# Autodesk Inventor assembly: ElevatorClaw
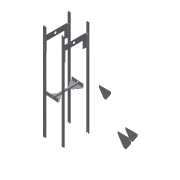
[picture p0: Inventor's stored thumbnail of the model, 180x180]
Saved by Autodesk Inventor 2015 (Build 190159000, 159)
## iProperties
Created: 2015-01-10
Part Number: ElevatorClaw
Document SubType Name: Assembly
Designer: Tanner
Author: Tanner
## Documents named in this file (8)
- C:\Users\Tanner\Documents\GitHub\FIRST-Team-1719-CAD-Team\2015 Robot CAD\Devices\Elevator and Claw\ElevatorClaw.iam
- C:\Users\Tanner\Documents\Inventor\ElevatorCAD\Kevin'sCustomUnistrut.ipt
- C:\Users\Tanner\Documents\Inventor\ElevatorCAD\Elevatorcarv2.iam
- C:\Users\Tanner\Documents\Inventor\ElevatorCAD\CarLbraket.ipt
- C:\Users\Tanner\Documents\Inventor\ElevatorCAD\elevbackplt.ipt
- C:\Users\Tanner\Documents\Inventor\ElevatorCAD\1 by 1 for the middle part of the elevator i dont even care anymore about names.ipt
- C:\Users\Tanner\Documents\Inventor\ElevatorCAD\super2.ipt
- C:\Users\Tanner\Documents\Inventor\ElevatorCAD\super4.ipt
## Components (21 placed, 7 different names)
1. Kevin'sCustomUnistrut:2 — Flush:17, Flush:27, Flush:28, Tangent:1, Mate:10
2. Kevin'sCustomUnistrut:3 — Flush:17, Flush:27, Flush:28, Tangent:2, Mate:11, Flush:48, Flush:51
3. Elevatorcarv2:1 [sub-assembly] — Flush:32, Mate:7, Flush:33, Tangent:2, Mate:11
4. Elevatorcarv2:3 [sub-assembly] — Mate:2, Flush:25, Flush:34, Tangent:1, Mate:10
5. CarLbraket:1 — Mate:2, Flush:25, Mate:4, Flush:34, Mate:9, Flush:37
6. CarLbraket:2 — Mate:4, Flush:32, Mate:7, Flush:33, Mate:8, Flush:35, Flush:36
7. elevbackplt:1 — Mate:8, Mate:9, Flush:35, Flush:36, Flush:37
8. Kevin'sCustomUnistrut:4
9. Kevin'sCustomUnistrut:5
10. Elevatorcarv2:4 [sub-assembly]
11. Elevatorcarv2:5 [sub-assembly]
12. CarLbraket:3
13. CarLbraket:4
14. elevbackplt:2
15. 1 by 1 for the middle part of the elevator i dont even care anymore about names:1 — Flush:48, Flush:49, Mate:19, Mate:20, Flush:50, Mate:21, Mate:22
16. super2:1 — Flush:50, Mate:21, Flush:51, Mate:22
17. super2:2 — Flush:49, Mate:19, Mate:20
18. super4:2
19. super4:4
20. super4:6
21. super4:9
## Relationships (46: Flush 24, Mate 18, Tangent 4)
- Flush:17: Kevin'sCustomUnistrut:2 ↔ Kevin'sCustomUnistrut:3
- Mate:2: Elevatorcarv2:3 ↔ CarLbraket:1
- Flush:25: Elevatorcarv2:3 ↔ CarLbraket:1
- Flush:27: Kevin'sCustomUnistrut:2 ↔ Kevin'sCustomUnistrut:3
- Flush:28: Kevin'sCustomUnistrut:2 ↔ Kevin'sCustomUnistrut:3
- Mate:4 (432.7144 mm): CarLbraket:1 ↔ CarLbraket:2
- Flush:32: Elevatorcarv2:1 ↔ CarLbraket:2
- Mate:7: Elevatorcarv2:1 ↔ CarLbraket:2
- Flush:33: Elevatorcarv2:1 ↔ CarLbraket:2
- Flush:34: Elevatorcarv2:3 ↔ CarLbraket:1
- Mate:8: CarLbraket:2 ↔ elevbackplt:1
- Mate:9: CarLbraket:1 ↔ elevbackplt:1
- Flush:35: CarLbraket:2 ↔ elevbackplt:1
- Flush:36 (-1.3462 mm): CarLbraket:2 ↔ elevbackplt:1
- Flush:37: CarLbraket:1 ↔ elevbackplt:1
- Tangent:1: Kevin'sCustomUnistrut:2 ↔ Elevatorcarv2:3
- Mate:10 (0.3683 mm): Kevin'sCustomUnistrut:2 ↔ Elevatorcarv2:3
- Tangent:2: Kevin'sCustomUnistrut:3 ↔ Elevatorcarv2:1
- Mate:11 (0.3683 mm): Kevin'sCustomUnistrut:3 ↔ Elevatorcarv2:1
- [Flush]: Kevin'sCustomUnistrut:4 ↔ Kevin'sCustomUnistrut:5
- [Mate]: Elevatorcarv2:5 ↔ CarLbraket:3
- [Flush]: Elevatorcarv2:5 ↔ CarLbraket:3
- [Flush]: Kevin'sCustomUnistrut:4 ↔ Kevin'sCustomUnistrut:5
- [Flush]: Kevin'sCustomUnistrut:4 ↔ Kevin'sCustomUnistrut:5
- [Mate] (432.7144 mm): CarLbraket:3 ↔ CarLbraket:4
- [Flush]: Elevatorcarv2:4 ↔ CarLbraket:4
- [Mate]: Elevatorcarv2:4 ↔ CarLbraket:4
- [Flush]: Elevatorcarv2:4 ↔ CarLbraket:4
- [Flush]: Elevatorcarv2:5 ↔ CarLbraket:3
- [Mate]: CarLbraket:4 ↔ elevbackplt:2
- [Mate]: CarLbraket:3 ↔ elevbackplt:2
- [Flush]: CarLbraket:4 ↔ elevbackplt:2
- [Flush] (-1.3462 mm): CarLbraket:4 ↔ elevbackplt:2
- [Flush]: CarLbraket:3 ↔ elevbackplt:2
- [Tangent]: Kevin'sCustomUnistrut:4 ↔ Elevatorcarv2:5
- [Mate] (0.3683 mm): Kevin'sCustomUnistrut:4 ↔ Elevatorcarv2:5
- [Tangent]: Kevin'sCustomUnistrut:5 ↔ Elevatorcarv2:4
- [Mate] (0.3683 mm): Kevin'sCustomUnistrut:5 ↔ Elevatorcarv2:4
- Flush:48: Kevin'sCustomUnistrut:3 ↔ 1 by 1 for the middle part of the elevator i dont even care anymore about names:1
- Flush:49: 1 by 1 for the middle part of the elevator i dont even care anymore about names:1 ↔ super2:2
- Mate:19: 1 by 1 for the middle part of the elevator i dont even care anymore about names:1 ↔ super2:2
- Mate:20: 1 by 1 for the middle part of the elevator i dont even care anymore about names:1 ↔ super2:2
- Flush:50: 1 by 1 for the middle part of the elevator i dont even care anymore about names:1 ↔ super2:1
- Mate:21: 1 by 1 for the middle part of the elevator i dont even care anymore about names:1 ↔ super2:1
- Flush:51: Kevin'sCustomUnistrut:3 ↔ super2:1
- Mate:22: 1 by 1 for the middle part of the elevator i dont even care anymore about names:1 ↔ super2:1
## Named parameters: d290_d285 = 0 mm, d291_d286 = 0.3683 mm, d292_d287 = 0 mm, d293_d288 = 0.3683 mm, d294_d257 = 0 mm, d295_d258 = 0 mm, d296_d261 = 0 mm, d297_d262 = 0 mm, d298_d263 = 432.7144 mm, d299_d270 = 0 mm, d300_d271 = 0 mm, d301_d274 = 0 mm, d302_d275 = 0 mm, d303_d276 = 0 mm, d304_d277 = 0 mm, d305_d278 = 0 mm, d306_d279 = -1.3462 mm, d307_d280 = 0 mm, d308_d181 = 0 mm
